# Autodesk Inventor assembly: DichroicCubeAssembly
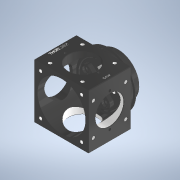
[picture p0: Inventor's stored thumbnail of the model, 180x180]
Saved by Autodesk Inventor 2020 (Build 240168000, 168)
## iProperties
Created: 2020-01-30
Part Number: DichroicCubeAssembly
Document SubType Name: Assembly
Designer: whgu0532
Author: whgu0532
## Documents named in this file (4)
- C:\Users\whgu0532\Documents\4Pi\4Pi-Oxford\DichroicCubeAssembly.iam
- C:\Users\whgu0532\Documents\4Pi\4Pi-Oxford\B4C_M.ipt
- C:\Users\whgu0532\Documents\4Pi\4Pi-Oxford\C4W.ipt
- C:\Users\whgu0532\Documents\4Pi\4Pi-Oxford\FFM1.ipt
## Components (3 placed, 3 different names)
1. B4C_M:1 — Mate:1, Mate:2, Mate:3, Rotational:2
2. C4W:1 — Rotational:2, Angle:1
3. FFM1:1 — Mate:1, Mate:2, Mate:3, Angle:1
## Relationships (5: Mate 3, RevoluteJoint 1, Angle 1)
- Mate:1: B4C_M:1 ↔ FFM1:1
- Mate:2: B4C_M:1 ↔ FFM1:1
- Mate:3: B4C_M:1 ↔ FFM1:1
- Rotational:2 [RevoluteJoint]: B4C_M:1 ↔ C4W:1
- Angle:1 (45 deg): C4W:1 ↔ FFM1:1
